# Autodesk Inventor assembly: Сборка1
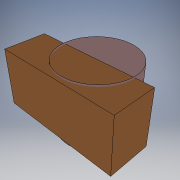
[picture p0: Inventor's stored thumbnail of the model, 180x180]
Saved by Autodesk Inventor 2019 (Build 230136000, 136)
## iProperties
Created: 2021-02-11
Part Number: Сборка1
Material: Типовые
Document SubType Name: Assembly
Designer: Kurbatova
Author: Kurbatova
## Documents named in this file (3)
- C:\Users\Kurbatova\source\LW2020\lw_2021\LW_SAPR\Сборки\Сборка1.iam
- C:\Users\Kurbatova\source\LW2020\lw_2021\LW_SAPR\Детали\Деталь2.ipt
- C:\Users\Kurbatova\source\LW2020\lw_2021\LW_SAPR\Детали\Деталь1.ipt
## Components (2 placed, 2 different names)
1. Деталь2:1 — Совмещение:1
2. Деталь1:1 — Совмещение:1
## Relationships (1: Mate 1)
- Совмещение:1 [Mate]: Деталь2:1 ↔ Деталь1:1
